# Autodesk Inventor assembly: ELECTRONICA AURA ENSAMBLADA
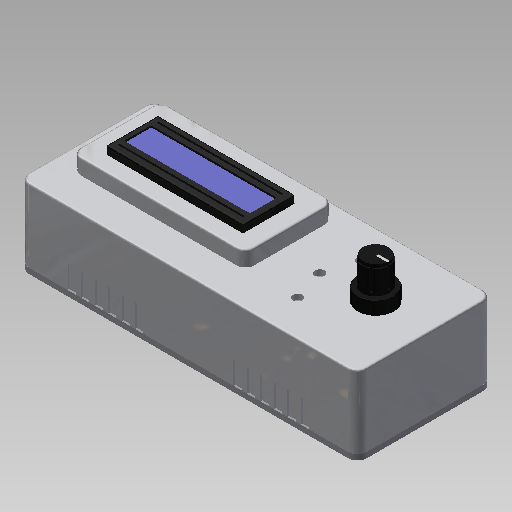
[picture p0: Inventor's stored thumbnail of the model, 512x512]
Saved by Autodesk Inventor 2019 (Build 230136000, 136)
## iProperties
Created: 2020-04-10
Part Number: ELECTRONICA AURA ENSAMBLADA
Material: Genérico
Document SubType Name: Assembly
Designer: Luis Pujol
Author: Luis Pujol
## Documents named in this file (6)
- C:\Users\Luis Pujol\Desktop\AURA MODELADO\ELECTRONICA\AURA ELECTRONICA\ELECTRONICA AURA ENSAMBLADA.iam
- C:\Users\Luis Pujol\Desktop\AURA MODELADO\ELECTRONICA\AURA ELECTRONICA\BASE INFERIOR.ipt
- C:\Users\Luis Pujol\Desktop\AURA MODELADO\ELECTRONICA\AURA ELECTRONICA\TAPA SUPEIOR.ipt
- C:\Users\Luis Pujol\Desktop\AURA MODELADO\ELECTRONICA\AURA ELECTRONICA\LCD_2x16.ipt
- C:\Users\Luis Pujol\Desktop\AURA MODELADO\ELECTRONICA\AURA ELECTRONICA\PANTALLA BASE.ipt
- C:\Users\Luis Pujol\Dropbox\TRABAJO\MECANICA\LIBRERIAS CAD MECANICA\PERILLA POTENCIOMETRO\Potentiometer knob.ipt
## Components (5 placed, 5 different names)
1. BASE INFERIOR:1 — Nivelación:1, Nivelación:2, Coincidencia:5
2. TAPA SUPEIOR:1 — Nivelación:1, Nivelación:2, Coincidencia:5, Coincidencia:9, Coincidencia:10, Coincidencia:11, Coincidencia:12, Coincidencia:13
3. LCD_2x16:1 — Coincidencia:6, Coincidencia:7, Coincidencia:8
4. PANTALLA BASE:1 — Coincidencia:6, Coincidencia:7, Coincidencia:8, Coincidencia:9, Coincidencia:10, Coincidencia:11
5. Potentiometer knob:1 — Coincidencia:12, Coincidencia:13
## Relationships (11: Mate 9, Flush 2)
- Nivelación:1 [Flush]: BASE INFERIOR:1 ↔ TAPA SUPEIOR:1
- Nivelación:2 [Flush]: BASE INFERIOR:1 ↔ TAPA SUPEIOR:1
- Coincidencia:5 [Mate]: BASE INFERIOR:1 ↔ TAPA SUPEIOR:1
- Coincidencia:6 [Mate]: LCD_2x16:1 ↔ PANTALLA BASE:1
- Coincidencia:7 [Mate]: LCD_2x16:1 ↔ PANTALLA BASE:1
- Coincidencia:8 [Mate]: LCD_2x16:1 ↔ PANTALLA BASE:1
- Coincidencia:9 [Mate]: TAPA SUPEIOR:1 ↔ PANTALLA BASE:1
- Coincidencia:10 [Mate]: TAPA SUPEIOR:1 ↔ PANTALLA BASE:1
- Coincidencia:11 [Mate]: TAPA SUPEIOR:1 ↔ PANTALLA BASE:1
- Coincidencia:12 [Mate] (2 mm): TAPA SUPEIOR:1 ↔ Potentiometer knob:1
- Coincidencia:13 [Mate]: TAPA SUPEIOR:1 ↔ Potentiometer knob:1
